# Autodesk Inventor assembly: cajas_V2_latest
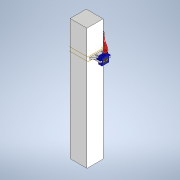
[picture p0: Inventor's stored thumbnail of the model, 180x180]
Saved by Autodesk Inventor 2020.3 (Build 243373000, 373)
## iProperties
Created: 2021-03-10
Part Number: cajas_V2_latest
Document SubType Name: Assembly
Designer: juanp
Author: juanp
## Documents named in this file (5)
- C:\Users\juanp\Desktop\Robocol\Nuevo EVA\V2\Cajas\cajas_V2_latest.iam
- C:\Users\juanp\Desktop\Robocol\Nuevo EVA\V2\Cajas\cajas_V2.ipt
- C:\Users\juanp\Desktop\Robocol\Nuevo EVA\V2\Cajas\Tapa_V2.ipt
- C:\Users\juanp\Desktop\Robocol\Nuevo EVA\V2\Cajas\Adaptador SG90.ipt
- C:\Users\juanp\Desktop\Robocol\Nuevo EVA\Recursos\Servo SG90\SG90 - Micro Servo 9g - Tower Pro.iam
## Components (4 placed, 4 different names)
1. cajas_V2:1 — Mate:3, Mate:5, Mate:6, Flush:1
2. Tapa_V2:1 — Flush:1, Mate:11
3. Adaptador SG90:1 — Mate:3, Mate:5, Mate:6, Mate:8, Mate:9, Mate:10
4. SG90 - Micro Servo 9g - Tower Pro:1 [sub-assembly] — Mate:8, Mate:9, Mate:10, Mate:11
## Relationships (8: Mate 7, Flush 1)
- Mate:3: cajas_V2:1 ↔ Adaptador SG90:1
- Mate:5: cajas_V2:1 ↔ Adaptador SG90:1
- Mate:6: cajas_V2:1 ↔ Adaptador SG90:1
- Mate:8: Adaptador SG90:1 ↔ SG90 - Micro Servo 9g - Tower Pro:1
- Mate:9: Adaptador SG90:1 ↔ SG90 - Micro Servo 9g - Tower Pro:1
- Mate:10: Adaptador SG90:1 ↔ SG90 - Micro Servo 9g - Tower Pro:1
- Flush:1: cajas_V2:1 ↔ Tapa_V2:1
- Mate:11: Tapa_V2:1 ↔ SG90 - Micro Servo 9g - Tower Pro:1
